# Autodesk Inventor assembly: Banh_xe
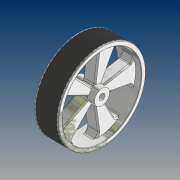
[picture p0: Inventor's stored thumbnail of the model, 180x180]
Saved by Autodesk Inventor 2021 (Build 250183000, 183)
## iProperties
Created: 2024-04-09
Part Number: Banh_xe
Document SubType Name: Assembly
Designer: Admin
Author: Admin
## Documents named in this file (3)
- C:\Users\Admin\Desktop\DO_AN_TOT_NGHIEP_2024\Mechanical\Design_in_3D\Library\Banh_xe.iam
- C:\Users\Admin\Desktop\DO_AN_TOT_NGHIEP_2024\Mechanical\Design_in_3D\Library\Lop_banh_xe.ipt
- C:\Users\Admin\Desktop\DO_AN_TOT_NGHIEP_2024\Mechanical\Design_in_3D\Library\Vanh_banh_xe.ipt
## Components (2 placed, 2 different names)
1. Lop_banh_xe:1 — Mate:1, Mate:2
2. Vanh_banh_xe:1 — Mate:1, Mate:2
## Relationships (2: Mate 2)
- Mate:1: Lop_banh_xe:1 ↔ Vanh_banh_xe:1
- Mate:2: Lop_banh_xe:1 ↔ Vanh_banh_xe:1
